# Autodesk Inventor assembly: Intake New Robot
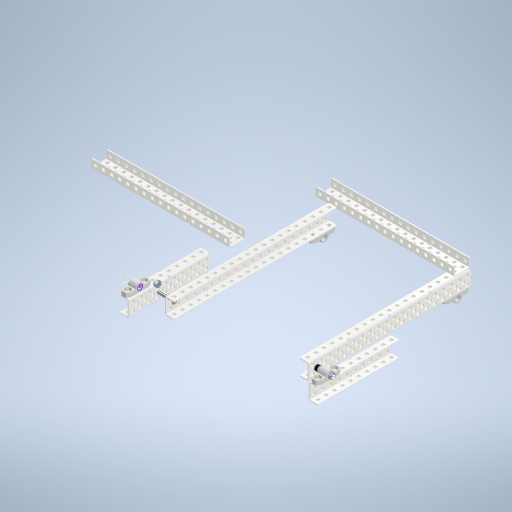
[picture p0: Inventor's stored thumbnail of the model, 512x512]
Saved by Autodesk Inventor 2023 (Build 270158000, 158)
## iProperties
Created: 2023-11-27
Part Number: Intake New Robot
Document SubType Name: Assembly
Designer: Robodox
Author: Robodox
## Documents named in this file (12)
- C:\Users\Robodox\Documents\GitHub\2023-599Z\BBotCAD\Intake New Robot.iam
- C:\Users\Robodox\Downloads\High Strength Pillow Block Bearing (276-8383).ipt
- C:\Users\Robodox\Documents\GitHub\2023-599Z\BBotCAD\VEX-CAD-Inventor-1.4.0\Structure\C Channel\Aluminum 1x2x1\Alu C 1x2x1x10.ipt
- C:\Users\Robodox\Documents\GitHub\2023-599Z\BBotCAD\VEX-CAD-Inventor-1.4.0\Structure\Hardware\Screw Steel - Star\SScrew Star Smooth 1.000.ipt
- C:\Users\Robodox\Documents\GitHub\2023-599Z\BBotCAD\VEX-CAD-Inventor-1.4.0\Structure\Hardware\Screw Steel - Star.ipt
- C:\Users\Robodox\Documents\GitHub\2023-599Z\BBotCAD\VEX-CAD-Inventor-1.4.0\Structure\Hardware\Nut Nylock.ipt
- C:\Users\Robodox\Documents\GitHub\2023-599Z\BBotCAD\VEX-CAD-Inventor-1.4.0\Structure\Hardware\Nut Keps.ipt
- C:\Users\Robodox\Documents\GitHub\2023-599Z\BBotCAD\VEX-CAD-Inventor-1.4.0\Motion\Spacers\Spacer Plastic\PSpacer 4.6.ipt
- C:\Users\Robodox\Documents\GitHub\2023-599Z\BBotCAD\VEX-CAD-Inventor-1.4.0\Motion\Spacers\Spacer Plastic.ipt
- C:\Users\Robodox\Documents\GitHub\2023-599Z\BBotCAD\VEX-CAD-Inventor-1.4.0\Structure\C Channel\Aluminum 1x2x1\Alu C 1x2x1x20.ipt
- C:\Users\Robodox\Documents\GitHub\2023-599Z\BBotCAD\VEX-CAD-Inventor-1.4.0\Structure\C Channel\Aluminum 1x2x1\Alu C 1x2x1x1.ipt
- C:\Users\Robodox\Documents\GitHub\2023-599Z\BBotCAD\VEX-CAD-Inventor-1.4.0\Structure\C Channel\Aluminum 1x2x1\Alu C 1x2x1x17.ipt
## Components (20 placed, 9 different names)
1. High Strength Pillow Block Bearing (276-8383):1 — Insert:3, Insert:4, Mate:1, Mate:2
2. Alu C 1x2x1x10:1 — Insert:3, Insert:4
3. Alu C 1x2x1x10:2 — Insert:6
4. SScrew Star Smooth 1.000:1 — Insert:5, Insert:21
5. Nut Nylock:1
6. Nut Nylock:2 — Insert:15
7. Nut Keps:2 — Insert:13
8. PSpacer 4.6:1 — Insert:21, Insert:22
9. Alu C 1x2x1x20:2 — Insert:5, Insert:16, Insert:17
10. High Strength Pillow Block Bearing (276-8383):2 — Insert:6, Mate:3
11. Nut Keps:3 — Insert:22
12. Alu C 1x2x1x1:1 — Mate:3, Insert:14
13. Alu C 1x2x1x1:2 — Mate:1, Mate:2
14. Alu C 1x2x1x20:4 — Insert:11, Insert:12, Insert:18, Insert:19, Insert:20
15. SScrew Star Smooth 1.000:2 — Insert:11, Insert:14, Insert:15
16. PSpacer 4.6:2 — Insert:12, Insert:13
17. High Strength Pillow Block Bearing (276-8383):3 — Insert:16, Insert:17
18. High Strength Pillow Block Bearing (276-8383):4 — Insert:18, Insert:19
19. Alu C 1x2x1x17:1
20. Alu C 1x2x1x17:2 — Insert:20
## Relationships (19: Insert 16, Mate 3)
- Insert:3: High Strength Pillow Block Bearing (276-8383):1 ↔ Alu C 1x2x1x10:1
- Insert:4: High Strength Pillow Block Bearing (276-8383):1 ↔ Alu C 1x2x1x10:1
- Insert:5: SScrew Star Smooth 1.000:1 ↔ Alu C 1x2x1x20:2
- Insert:6: Alu C 1x2x1x10:2 ↔ High Strength Pillow Block Bearing (276-8383):2
- Mate:1: High Strength Pillow Block Bearing (276-8383):1 ↔ Alu C 1x2x1x1:2
- Mate:2: High Strength Pillow Block Bearing (276-8383):1 ↔ Alu C 1x2x1x1:2
- Insert:11: Alu C 1x2x1x20:4 ↔ SScrew Star Smooth 1.000:2
- Insert:12: Alu C 1x2x1x20:4 ↔ PSpacer 4.6:2
- Insert:13: Nut Keps:2 ↔ PSpacer 4.6:2
- Mate:3: High Strength Pillow Block Bearing (276-8383):2 ↔ Alu C 1x2x1x1:1
- Insert:14 (-15.494 mm): Alu C 1x2x1x1:1 ↔ SScrew Star Smooth 1.000:2
- Insert:15 (-3.048 mm): Nut Nylock:2 ↔ SScrew Star Smooth 1.000:2
- Insert:16: Alu C 1x2x1x20:2 ↔ High Strength Pillow Block Bearing (276-8383):3
- Insert:17: Alu C 1x2x1x20:2 ↔ High Strength Pillow Block Bearing (276-8383):3
- Insert:18: Alu C 1x2x1x20:4 ↔ High Strength Pillow Block Bearing (276-8383):4
- Insert:19: Alu C 1x2x1x20:4 ↔ High Strength Pillow Block Bearing (276-8383):4
- Insert:20: Alu C 1x2x1x20:4 ↔ Alu C 1x2x1x17:2
- Insert:21 (-23.8252 mm): SScrew Star Smooth 1.000:1 ↔ PSpacer 4.6:1
- Insert:22: PSpacer 4.6:1 ↔ Nut Keps:3
